# Autodesk Inventor assembly: BodyStructure
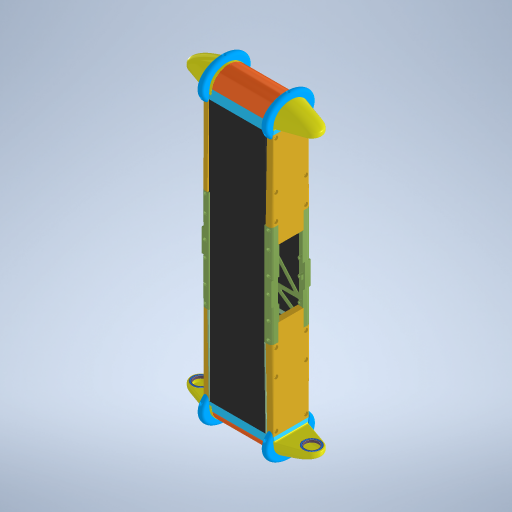
[picture p0: Inventor's stored thumbnail of the model, 512x512]
Saved by Autodesk Inventor 2023 (Build 270158000, 158)
## iProperties
Created: 2022-01-14
Part Number: BodyStructure
Document SubType Name: Assembly
Designer: Jochen
Author: Jochen
## Documents named in this file (11)
- D:\Projects\Lisbeth\CAD\BodyStructure.iam
- D:\Projects\Lisbeth\CAD\Body\BodyStructure Side.ipt
- D:\Projects\Lisbeth\CAD\Body\BodyStructure HipSupport.ipt
- D:\Projects\Lisbeth\CAD\Body\BodyStructure Front.ipt
- D:\Projects\Lisbeth\CAD\Body\BodyStructure Centre Top.ipt
- D:\Projects\Lisbeth\CAD\Body\BodyStructure Plate.ipt
- D:\Projects\Lisbeth\CAD\Common\Bearing\bearing_27_20_4 s61704-2rsr.ipt
- D:\Projects\Lisbeth\CAD\Body\BodyCover.ipt
- D:\Projects\Lisbeth\CAD\Common\Battery\Battery Pack.ipt
- D:\Projects\Lisbeth\CAD\Body\BodyStructure Centre Bottom.ipt
- D:\Projects\Lisbeth\CAD\Body\BodyDampener.ipt
## Components (25 placed, 9 different names)
1. BodyStructure Side:1 — Mate:73, Mate:89, Mate:100, Mate:102, Mate:108, Flush:7
2. BodyStructure Side:2 — Mate:74, Mate:107, Mate:109, Mate:110, Mate:111, Flush:8
3. BodyHipSupport:1 — Mate:38, Mate:39, Mate:76, Mate:77
4. BodyHipSupport:2 — Mate:44, Mate:45, Mate:78, Mate:79
5. Body Structure Centre Top:2 — Mate:46, Mate:95, Mate:115, Mate:116
6. BodyStructure Side:3 — Mate:20, Mate:46, Mate:87, Mate:114, Flush:6
7. BodyStructure Side:4 — Mate:88, Mate:101, Mate:112, Mate:115, Flush:5
8. BodyStructure Front:2 — Mate:20, Mate:21, Mate:22, Mate:23, Mate:24, Mate:87, Mate:88, Mate:99, Mate:105, Mate:106, Mate:112, Mate:114, Mate:129, Mate:130, Mate:131, Mate:132
9. BodyHipSupport:3 — Mate:23, Mate:24, Mate:42, Mate:43
10. BodyHipSupport:4 — Mate:21, Mate:22, Mate:40, Mate:41
11. bearing_27_20_4 s61704-2rsr:1 — Mate:38, Mate:39
12. bearing_27_20_4 s61704-2rsr:2 — Mate:44, Mate:45
13. bearing_27_20_4 s61704-2rsr:3 — Mate:40, Mate:41
14. bearing_27_20_4 s61704-2rsr:4 — Mate:42, Mate:43
15. BodyCover:1 — Mate:103, Mate:113
16. BodyCover:2 — Mate:95, Mate:99, Mate:116
17. Battery Pack 59x31x21:1
18. BodyStructure Front:3 — Mate:73, Mate:74, Mate:76, Mate:77, Mate:78, Mate:79, Mate:105, Mate:106, Mate:107, Mate:108, Mate:133, Mate:134, Mate:135, Mate:136
19. Body Structure Centre:7 — Mate:89, Mate:109
20. Body Structure Centre Top:1 — Mate:100, Mate:101, Mate:102, Mate:103, Mate:113
21. Body Structure Centre:9 — Mate:110, Mate:111
22. BodyDampener:1 — Mate:129, Mate:130, Flush:5
23. BodyDampener:2 — Mate:131, Mate:132, Flush:6
24. BodyDampener:3 — Mate:133, Mate:136, Flush:7
25. BodyDampener:4 — Mate:134, Mate:135, Flush:8
## Relationships (53: Mate 49, Flush 4)
- Mate:20: BodyStructure Side:3 ↔ BodyStructure Front:2
- Mate:21: BodyStructure Front:2 ↔ BodyHipSupport:4
- Mate:22: BodyStructure Front:2 ↔ BodyHipSupport:4
- Mate:23: BodyStructure Front:2 ↔ BodyHipSupport:3
- Mate:24: BodyStructure Front:2 ↔ BodyHipSupport:3
- Mate:38: BodyHipSupport:1 ↔ bearing_27_20_4 s61704-2rsr:1
- Mate:39: BodyHipSupport:1 ↔ bearing_27_20_4 s61704-2rsr:1
- Mate:40: BodyHipSupport:4 ↔ bearing_27_20_4 s61704-2rsr:3
- Mate:41: BodyHipSupport:4 ↔ bearing_27_20_4 s61704-2rsr:3
- Mate:42: BodyHipSupport:3 ↔ bearing_27_20_4 s61704-2rsr:4
- Mate:43: BodyHipSupport:3 ↔ bearing_27_20_4 s61704-2rsr:4
- Mate:44: BodyHipSupport:2 ↔ bearing_27_20_4 s61704-2rsr:2
- Mate:45: BodyHipSupport:2 ↔ bearing_27_20_4 s61704-2rsr:2
- Mate:46: Body Structure Centre Top:2 ↔ BodyStructure Side:3
- Mate:73: BodyStructure Side:1 ↔ BodyStructure Front:3
- Mate:74: BodyStructure Side:2 ↔ BodyStructure Front:3
- Mate:76: BodyHipSupport:1 ↔ BodyStructure Front:3
- Mate:77: BodyHipSupport:1 ↔ BodyStructure Front:3
- Mate:78: BodyHipSupport:2 ↔ BodyStructure Front:3
- Mate:79: BodyHipSupport:2 ↔ BodyStructure Front:3
- Mate:87: BodyStructure Side:3 ↔ BodyStructure Front:2
- Mate:88: BodyStructure Side:4 ↔ BodyStructure Front:2
- Mate:89: BodyStructure Side:1 ↔ Body Structure Centre:7
- Mate:95: Body Structure Centre Top:2 ↔ BodyCover:2
- Mate:99: BodyStructure Front:2 ↔ BodyCover:2
- Mate:100: BodyStructure Side:1 ↔ Body Structure Centre Top:1
- Mate:101: BodyStructure Side:4 ↔ Body Structure Centre Top:1
- Mate:102: BodyStructure Side:1 ↔ Body Structure Centre Top:1
- Mate:103: BodyCover:1 ↔ Body Structure Centre Top:1
- Mate:105: BodyStructure Front:2 ↔ BodyStructure Front:3
- Mate:106: BodyStructure Front:2 ↔ BodyStructure Front:3
- Mate:107: BodyStructure Side:2 ↔ BodyStructure Front:3
- Mate:108: BodyStructure Side:1 ↔ BodyStructure Front:3
- Mate:109: BodyStructure Side:2 ↔ Body Structure Centre:7
- Mate:110: BodyStructure Side:2 ↔ Body Structure Centre:9
- Mate:111: BodyStructure Side:2 ↔ Body Structure Centre:9
- Mate:112: BodyStructure Side:4 ↔ BodyStructure Front:2
- Mate:113: BodyCover:1 ↔ Body Structure Centre Top:1
- Mate:114: BodyStructure Side:3 ↔ BodyStructure Front:2
- Mate:115: Body Structure Centre Top:2 ↔ BodyStructure Side:4
- Mate:116: Body Structure Centre Top:2 ↔ BodyCover:2
- Mate:129: BodyStructure Front:2 ↔ BodyDampener:1
- Mate:130: BodyStructure Front:2 ↔ BodyDampener:1
- Flush:5: BodyStructure Side:4 ↔ BodyDampener:1
- Mate:131: BodyStructure Front:2 ↔ BodyDampener:2
- Mate:132: BodyStructure Front:2 ↔ BodyDampener:2
- Flush:6: BodyStructure Side:3 ↔ BodyDampener:2
- Mate:133: BodyStructure Front:3 ↔ BodyDampener:3
- Mate:134: BodyStructure Front:3 ↔ BodyDampener:4
- Mate:135: BodyStructure Front:3 ↔ BodyDampener:4
- Mate:136: BodyStructure Front:3 ↔ BodyDampener:3
- Flush:7: BodyStructure Side:1 ↔ BodyDampener:3
- Flush:8: BodyStructure Side:2 ↔ BodyDampener:4
